# Autodesk Inventor assembly: Vert - 1in
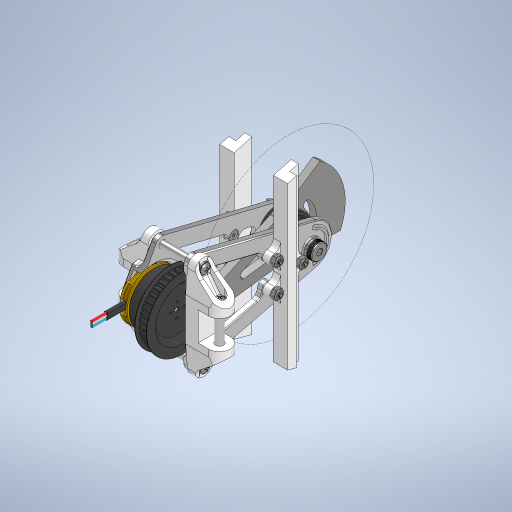
[picture p0: Inventor's stored thumbnail of the model, 512x512]
Saved by Autodesk Inventor 2023.2 (Build 272271000, 271)
## iProperties
Created: 2023-07-17
Part Number: Vert - 1in
Document SubType Name: Assembly
Designer: Nathan Cai
Mass: 648.971 g
Surface Area: 1316.81 cm^2
Volume: 214.133 cm^3
Density: 3.03069 g/cm^3
Author: Nathan Cai
## Documents named in this file (24)
- E:\Documents\Inventor\Law - V1.0\Vert - 1in\Vert - 1in.iam
- E:\Documents\Inventor\Law - V1.0\Vert - 1in\FEICHAO BE4108 380KV\FEICHAO BE4108 380KV.iam
- E:\Documents\Inventor\Law - V1.0\Vert - 1in\Blade (Bar 3).ipt
- E:\Documents\Inventor\Law - V1.0\Vert - 1in\Upright - Motor.ipt
- E:\Documents\Inventor\Law - V1.0\Standoff 1in.ipt
- E:\Documents\Inventor\Law - V1.0\Vert - 1in\Leg.ipt
- E:\Documents\Inventor\Law - V1.0\Vert - 1in\Upright - Blank.ipt
- E:\Documents\Inventor\Law - V1.0\Vert - 1in\91259A628_Alloy Steel Shoulder Screw.ipt
- E:\Documents\Inventor\Law - V1.0\Vert - 1in\90630A121_High-Strength Steel Nylon-Insert Locknut.ipt
- E:\Documents\Inventor\Law - V1.0\Vertical Weapon Assembly (Type A)\XL Pulley 18T .25in Wd.ipt
- E:\Documents\Inventor\Law - V1.0\Vertical Weapon Assembly (Type A)\Spacer 3-8x .125.ipt
- E:\Documents\Inventor\Law - V1.0\Vert - 1in\Needle Bearings.ipt
- E:\Documents\Inventor\Law - V1.0\Vert - 1in\5905K497_Needle-Roller Bearing (1).ipt
- E:\Documents\Inventor\Law - V1.0\Vert - 1in\XL Pulley 36T .375in Wd.ipt
- E:\Documents\Inventor\Law - V1.0\Vert - 1in\6-32 x 5-8.ipt
- E:\Documents\Inventor\Law - V1.0\Vert - 1in\6-32 Nylock.ipt
- E:\Documents\Inventor\Content Center Files\R2023\en-US\ISO 4762(2)\ISO 4762 - M3 x 8ISO.ipt
- E:\Documents\Inventor\Law - V1.0\Vert - 1in\Bracket.ipt
- E:\Documents\Inventor\Law - V1.0\Vert - 1in\Standoff 1.5in.ipt
- E:\Documents\Inventor\Content Center Files\R2023\en-US\ANSI B18.22.1\ANSI B18.22.1 - No. 6 - Type A.ipt
- E:\Documents\Inventor\Content Center Files\R2023\en-US\ANSI B18.6.3(27)\ANSI B18.6.3 - 6-32 UNC - 0.375(11).ipt
- E:\Documents\Inventor\Content Center Files\R2023\en-US\ANSI B18.22.1\ANSI B18.22.1 - No. 6 - narrow - Type B.ipt
- E:\Documents\Inventor\Content Center Files\R2023\en-US\ANSI B18.6.3(27)\ANSI B18.6.3 - 6-32 UNC - 0.75(11).ipt
- E:\Documents\Inventor\Law - V1.0\Vert - 1in\Bracket - Clear.ipt
## Components (53 placed, 23 different names)
1. FEICHAO BE4108 380KV:1 [sub-assembly] — Mate:1, Mate:2, Mate:11, Mate:43, Mate:44
2. Blade (Bar 3):1 — Mate:3, Mate:29, Mate:30, Mate:37, Mate:38, Mate:39, Mate:41
3. Upright - Motor:1 — Mate:1, Mate:2, Mate:3, Mate:4, Mate:5, Mate:6, Mate:7, Mate:11, Mate:12, Mate:13, Mate:14, Mate:24, Mate:32, Mate:58, Mate:59, Mate:60, Mate:61, Mate:62, Mate:63, Mate:70, Mate:71, Mate:72, Mate:73, Mate:74, Mate:75, Mate:76, Mate:77, Mate:78, Mate:79, Mate:101
4. Upright - Blank:1 — Mate:15, Mate:16, Mate:17, Mate:18, Mate:19, Mate:20, Mate:22, Mate:23, Mate:34, Mate:45, Mate:46, Mate:47, Mate:48, Mate:49, Mate:50, Mate:51, Mate:100
5. Standoff 1in:1 — Mate:5, Mate:7, Mate:15, Mate:16
6. Standoff 1in:2 — Mate:4, Mate:6, Mate:17
7. Leg:1 — Mate:12, Mate:13, Mate:14, Mate:64, Mate:65, Mate:66
8. Leg:2 — Mate:18, Mate:19, Mate:20, Mate:52, Mate:53, Mate:54
9. 91259A628_Alloy Steel Shoulder Screw:1 — Mate:22, Mate:23, Mate:25, Mate:31, Mate:33, Mate:36
10. 90630A121_High-Strength Steel Nylon-Insert Locknut:1 — Mate:24, Mate:25
11. XL Pulley 18T .25in Wd:1 — Mate:36, Mate:37, Mate:38, Mate:40, Flush:2, Flush:3
12. XL Pulley 36T .375in Wd:1 — Flush:3, Mate:43, Mate:44
13. Spacer 3-8x .125:1 — Mate:29, Mate:30, Mate:39, Flush:1, Mate:42
14. Needle Bearings:1 — Mate:31, Mate:32, Mate:42
15. Needle Bearings:2 — Mate:33, Mate:34
16. 5905K497_Needle-Roller Bearing (1):1 — Mate:41, Flush:1
17. 5905K497_Needle-Roller Bearing (1):2 — Mate:40, Flush:2
18. ISO 4762 M3 x 8:1 — Mate:70, Mate:71
19. ISO 4762 M3 x 8:2 — Mate:72, Mate:73
20. ISO 4762 M3 x 8:3 — Mate:74, Mate:75
21. ISO 4762 M3 x 8:4 — Mate:76, Mate:77
22. 6-32 x 5-8:1 — Mate:47, Mate:49, Mate:50, Mate:55
23. 6-32 x 5-8:2 — Mate:46, Mate:48, Mate:56
24. 6-32 x 5-8:3 — Mate:45, Mate:51, Mate:57
25. 6-32 x 5-8:4 — Mate:59, Mate:63, Mate:67
26. 6-32 x 5-8:5 — Mate:58, Mate:61, Mate:68
27. 6-32 x 5-8:6 — Mate:60, Mate:62, Mate:69
28. 6-32 Nylock:1 — Mate:64, Mate:67
29. 6-32 Nylock:2 — Mate:66, Mate:69
30. 6-32 Nylock:3 — Mate:65, Mate:68
31. 6-32 Nylock:4 — Mate:52, Mate:56
32. 6-32 Nylock:5 — Mate:53, Mate:57
33. 6-32 Nylock:6 — Mate:54, Mate:55
34. Bracket:2 — Mate:78, Mate:79, Mate:80, Flush:4, Mate:85, Mate:86, Mate:87, Mate:88, Flush:6, Mate:99, Mate:101
35. Standoff 1.5in:1 — Mate:80, Flush:4, Mate:81, Mate:82, Mate:83, Mate:84
36. Plain Washer (Inch) No. 6 - Type A:1 — Mate:81, Mate:82, Insert:1
37. Cross Recessed Truss Head Machine Screw - Type I - Inch No. 6 - 32 - 3/8:1 — Insert:1
38. Plain Washer (Inch) No. 6 - Type A:2 — Mate:83, Mate:84, Insert:2
39. Cross Recessed Truss Head Machine Screw - Type I - Inch No. 6 - 32 - 3/8:2 — Insert:2
40. Plain Washer (Inch) No. 6 - narrow - Type B:1 — Mate:85, Mate:86, Insert:3
41. Cross Recessed Truss Head Machine Screw - Type I - Inch No. 6 - 32 - 3/4:1 — Insert:3
42. Plain Washer (Inch) No. 6 - narrow - Type B:2 — Mate:87, Mate:88, Insert:4
43. Cross Recessed Truss Head Machine Screw - Type I - Inch No. 6 - 32 - 3/4:2 — Insert:4
44. Standoff 1.5in:2 — Mate:90, Flush:5, Mate:91, Mate:92, Mate:93, Mate:94
45. Bracket - Clear:1 — Mate:90, Flush:5, Mate:95, Mate:96, Mate:97, Mate:98, Flush:6, Mate:99, Mate:100
46. Plain Washer (Inch) No. 6 - Type A:3 — Mate:91, Mate:92, Insert:5
47. Cross Recessed Truss Head Machine Screw - Type I - Inch No. 6 - 32 - 3/8:3 — Insert:5
48. Plain Washer (Inch) No. 6 - Type A:4 — Mate:93, Mate:94, Insert:6
49. Cross Recessed Truss Head Machine Screw - Type I - Inch No. 6 - 32 - 3/8:4 — Insert:6
50. Plain Washer (Inch) No. 6 - Type A:5 — Mate:95, Mate:96, Insert:7
51. Cross Recessed Truss Head Machine Screw - Type I - Inch No. 6 - 32 - 3/4:3 — Insert:7
52. Plain Washer (Inch) No. 6 - Type A:6 — Mate:97, Mate:98, Insert:8
53. Cross Recessed Truss Head Machine Screw - Type I - Inch No. 6 - 32 - 3/4:4 — Insert:8
## Relationships (106: Mate 92, Insert 8, Flush 6)
- Mate:1: FEICHAO BE4108 380KV:1 ↔ Upright - Motor:1
- Mate:2: FEICHAO BE4108 380KV:1 ↔ Upright - Motor:1
- Mate:3: Blade (Bar 3):1 ↔ Upright - Motor:1
- Mate:4: Upright - Motor:1 ↔ Standoff 1in:2
- Mate:5: Upright - Motor:1 ↔ Standoff 1in:1
- Mate:6: Upright - Motor:1 ↔ Standoff 1in:2
- Mate:7: Upright - Motor:1 ↔ Standoff 1in:1
- Mate:11: FEICHAO BE4108 380KV:1 ↔ Upright - Motor:1
- Mate:12: Upright - Motor:1 ↔ Leg:1
- Mate:13: Upright - Motor:1 ↔ Leg:1
- Mate:14: Upright - Motor:1 ↔ Leg:1
- Mate:15: Upright - Blank:1 ↔ Standoff 1in:1
- Mate:16: Upright - Blank:1 ↔ Standoff 1in:1
- Mate:17: Upright - Blank:1 ↔ Standoff 1in:2
- Mate:18: Upright - Blank:1 ↔ Leg:2
- Mate:19: Upright - Blank:1 ↔ Leg:2
- Mate:20: Upright - Blank:1 ↔ Leg:2
- Mate:22: Upright - Blank:1 ↔ 91259A628_Alloy Steel Shoulder Screw:1
- Mate:23: Upright - Blank:1 ↔ 91259A628_Alloy Steel Shoulder Screw:1
- Mate:24: Upright - Motor:1 ↔ 90630A121_High-Strength Steel Nylon-Insert Locknut:1
- Mate:25: 91259A628_Alloy Steel Shoulder Screw:1 ↔ 90630A121_High-Strength Steel Nylon-Insert Locknut:1
- Mate:29: Blade (Bar 3):1 ↔ Spacer 3-8x .125:1
- Mate:30: Blade (Bar 3):1 ↔ Spacer 3-8x .125:1
- Mate:31: 91259A628_Alloy Steel Shoulder Screw:1 ↔ Needle Bearings:1
- Mate:32: Upright - Motor:1 ↔ Needle Bearings:1
- Mate:33: 91259A628_Alloy Steel Shoulder Screw:1 ↔ Needle Bearings:2
- Mate:34: Upright - Blank:1 ↔ Needle Bearings:2
- Mate:36: 91259A628_Alloy Steel Shoulder Screw:1 ↔ XL Pulley 18T .25in Wd:1
- Mate:37: Blade (Bar 3):1 ↔ XL Pulley 18T .25in Wd:1
- Mate:38: Blade (Bar 3):1 ↔ XL Pulley 18T .25in Wd:1
- Mate:39: Blade (Bar 3):1 ↔ Spacer 3-8x .125:1
- Mate:40: XL Pulley 18T .25in Wd:1 ↔ 5905K497_Needle-Roller Bearing (1):2
- Mate:41: Blade (Bar 3):1 ↔ 5905K497_Needle-Roller Bearing (1):1
- Flush:1: Spacer 3-8x .125:1 ↔ 5905K497_Needle-Roller Bearing (1):1
- Flush:2: XL Pulley 18T .25in Wd:1 ↔ 5905K497_Needle-Roller Bearing (1):2
- Mate:42: Spacer 3-8x .125:1 ↔ Needle Bearings:1
- Flush:3: XL Pulley 18T .25in Wd:1 ↔ XL Pulley 36T .375in Wd:1
- Mate:43: FEICHAO BE4108 380KV:1 ↔ XL Pulley 36T .375in Wd:1
- Mate:44: FEICHAO BE4108 380KV:1 ↔ XL Pulley 36T .375in Wd:1
- Mate:45: Upright - Blank:1 ↔ 6-32 x 5-8:3
- Mate:46: Upright - Blank:1 ↔ 6-32 x 5-8:2
- Mate:47: Upright - Blank:1 ↔ 6-32 x 5-8:1
- Mate:48: Upright - Blank:1 ↔ 6-32 x 5-8:2
- Mate:49: Upright - Blank:1 ↔ 6-32 x 5-8:1
- Mate:50: Upright - Blank:1 ↔ 6-32 x 5-8:1
- Mate:51: Upright - Blank:1 ↔ 6-32 x 5-8:3
- Mate:52: Leg:2 ↔ 6-32 Nylock:4
- Mate:53: Leg:2 ↔ 6-32 Nylock:5
- Mate:54: Leg:2 ↔ 6-32 Nylock:6
- Mate:55: 6-32 x 5-8:1 ↔ 6-32 Nylock:6
- Mate:56: 6-32 x 5-8:2 ↔ 6-32 Nylock:4
- Mate:57: 6-32 x 5-8:3 ↔ 6-32 Nylock:5
- Mate:58: Upright - Motor:1 ↔ 6-32 x 5-8:5
- Mate:59: Upright - Motor:1 ↔ 6-32 x 5-8:4
- Mate:60: Upright - Motor:1 ↔ 6-32 x 5-8:6
- Mate:61: Upright - Motor:1 ↔ 6-32 x 5-8:5
- Mate:62: Upright - Motor:1 ↔ 6-32 x 5-8:6
- Mate:63: Upright - Motor:1 ↔ 6-32 x 5-8:4
- Mate:64: Leg:1 ↔ 6-32 Nylock:1
- Mate:65: Leg:1 ↔ 6-32 Nylock:3
- Mate:66: Leg:1 ↔ 6-32 Nylock:2
- Mate:67: 6-32 x 5-8:4 ↔ 6-32 Nylock:1
- Mate:68: 6-32 x 5-8:5 ↔ 6-32 Nylock:3
- Mate:69: 6-32 x 5-8:6 ↔ 6-32 Nylock:2
- Mate:70: Upright - Motor:1 ↔ ISO 4762 M3 x 8:1
- Mate:71: Upright - Motor:1 ↔ ISO 4762 M3 x 8:1
- Mate:72: Upright - Motor:1 ↔ ISO 4762 M3 x 8:2
- Mate:73: Upright - Motor:1 ↔ ISO 4762 M3 x 8:2
- Mate:74: Upright - Motor:1 ↔ ISO 4762 M3 x 8:3
- Mate:75: Upright - Motor:1 ↔ ISO 4762 M3 x 8:3
- Mate:76: Upright - Motor:1 ↔ ISO 4762 M3 x 8:4
- Mate:77: Upright - Motor:1 ↔ ISO 4762 M3 x 8:4
- Mate:78: Upright - Motor:1 ↔ Bracket:2
- Mate:79: Upright - Motor:1 ↔ Bracket:2
- Mate:80: Bracket:2 ↔ Standoff 1.5in:1
- Flush:4: Bracket:2 ↔ Standoff 1.5in:1
- Mate:81: Standoff 1.5in:1 ↔ Plain Washer (Inch) No. 6 - Type A:1
- Mate:82: Standoff 1.5in:1 ↔ Plain Washer (Inch) No. 6 - Type A:1
- Insert:1: Plain Washer (Inch) No. 6 - Type A:1 ↔ Cross Recessed Truss Head Machine Screw - Type I - Inch No. 6 - 32 - 3/8:1
- Mate:83: Standoff 1.5in:1 ↔ Plain Washer (Inch) No. 6 - Type A:2
- Mate:84: Standoff 1.5in:1 ↔ Plain Washer (Inch) No. 6 - Type A:2
- Insert:2: Plain Washer (Inch) No. 6 - Type A:2 ↔ Cross Recessed Truss Head Machine Screw - Type I - Inch No. 6 - 32 - 3/8:2
- Mate:85: Bracket:2 ↔ Plain Washer (Inch) No. 6 - narrow - Type B:1
- Mate:86: Bracket:2 ↔ Plain Washer (Inch) No. 6 - narrow - Type B:1
- Mate:87: Bracket:2 ↔ Plain Washer (Inch) No. 6 - narrow - Type B:2
- Mate:88: Bracket:2 ↔ Plain Washer (Inch) No. 6 - narrow - Type B:2
- Insert:3: Plain Washer (Inch) No. 6 - narrow - Type B:1 ↔ Cross Recessed Truss Head Machine Screw - Type I - Inch No. 6 - 32 - 3/4:1
- Insert:4: Plain Washer (Inch) No. 6 - narrow - Type B:2 ↔ Cross Recessed Truss Head Machine Screw - Type I - Inch No. 6 - 32 - 3/4:2
- Mate:90: Standoff 1.5in:2 ↔ Bracket - Clear:1
- Flush:5: Standoff 1.5in:2 ↔ Bracket - Clear:1
- Mate:91: Standoff 1.5in:2 ↔ Plain Washer (Inch) No. 6 - Type A:3
- Mate:92: Standoff 1.5in:2 ↔ Plain Washer (Inch) No. 6 - Type A:3
- Insert:5: Plain Washer (Inch) No. 6 - Type A:3 ↔ Cross Recessed Truss Head Machine Screw - Type I - Inch No. 6 - 32 - 3/8:3
- Mate:93: Standoff 1.5in:2 ↔ Plain Washer (Inch) No. 6 - Type A:4
- Mate:94: Standoff 1.5in:2 ↔ Plain Washer (Inch) No. 6 - Type A:4
- Insert:6: Plain Washer (Inch) No. 6 - Type A:4 ↔ Cross Recessed Truss Head Machine Screw - Type I - Inch No. 6 - 32 - 3/8:4
- Mate:95: Bracket - Clear:1 ↔ Plain Washer (Inch) No. 6 - Type A:5
- Mate:96: Bracket - Clear:1 ↔ Plain Washer (Inch) No. 6 - Type A:5
- Mate:97: Bracket - Clear:1 ↔ Plain Washer (Inch) No. 6 - Type A:6
- Mate:98: Bracket - Clear:1 ↔ Plain Washer (Inch) No. 6 - Type A:6
- Insert:7: Plain Washer (Inch) No. 6 - Type A:5 ↔ Cross Recessed Truss Head Machine Screw - Type I - Inch No. 6 - 32 - 3/4:3
- Insert:8: Plain Washer (Inch) No. 6 - Type A:6 ↔ Cross Recessed Truss Head Machine Screw - Type I - Inch No. 6 - 32 - 3/4:4
- Flush:6: Bracket:2 ↔ Bracket - Clear:1
- Mate:99: Bracket:2 ↔ Bracket - Clear:1
- Mate:100: Upright - Blank:1 ↔ Bracket - Clear:1
- Mate:101: Upright - Motor:1 ↔ Bracket:2
